# Autodesk Inventor assembly: support
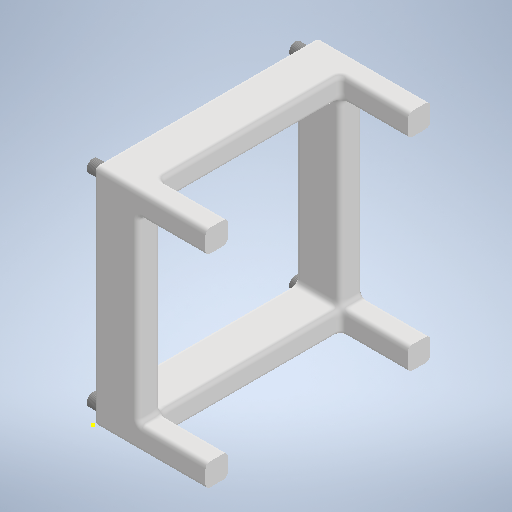
[picture p0: Inventor's stored thumbnail of the model, 512x512]
Saved by Autodesk Inventor 2025.2 (Build 292293000, 293)
## iProperties
Created: 2025-02-15
Part Number: support
Document SubType Name: Assembly
Designer: antoi
Author: antoi
## Documents named in this file (3)
- C:\Users\antoi\Documents\Henallux_24_25\Q2\proj\prototype\support.iam
- C:\Users\antoi\Documents\Henallux_24_25\Q2\proj\prototype\Pièce1.ipt
- C:\Users\antoi\Documents\Henallux_24_25\Q2\proj\prototype\vis.ipt
## Components (5 placed, 2 different names)
1. Pièce1:1 — Affleurement:1, Placage:1, Placage:2, Placage:3, Placage:4, Affleurement:2, Affleurement:3, Affleurement:4, Affleurement:5
2. vis:1 — Placage:3, Affleurement:2
3. vis:2 — Placage:4, Affleurement:3
4. vis:3 — Placage:2, Affleurement:5
5. vis:4 — Placage:1, Affleurement:4
## Relationships (9: Flush 5, Mate 4)
- Affleurement:1 [Flush] (-5 mm): Pièce1:1
- Placage:1 [Mate]: Pièce1:1 ↔ vis:4
- Placage:2 [Mate]: Pièce1:1 ↔ vis:3
- Placage:3 [Mate]: Pièce1:1 ↔ vis:1
- Placage:4 [Mate]: Pièce1:1 ↔ vis:2
- Affleurement:2 [Flush] (-5 mm): Pièce1:1 ↔ vis:1
- Affleurement:3 [Flush] (-5 mm): Pièce1:1 ↔ vis:2
- Affleurement:4 [Flush] (5 mm): Pièce1:1 ↔ vis:4
- Affleurement:5 [Flush] (-5 mm): Pièce1:1 ↔ vis:3
